# Autodesk Inventor assembly: Ensamble1
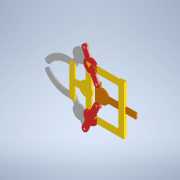
[picture p0: Inventor's stored thumbnail of the model, 180x180]
Saved by Autodesk Inventor 2021 (Build 250183000, 183)
## iProperties
Created: 2022-11-01
Part Number: Ensamble1
Document SubType Name: Assembly
Designer: USUARIO
Author: USUARIO
## Documents named in this file (6)
- C:\Users\USUARIO\Documents\Semestre8\Robótica\Proyecto-Rob\Piezas\Ensamble1.iam
- C:\Users\USUARIO\Documents\Semestre8\Robótica\Proyecto-Rob\Piezas\BaseGripper.ipt
- C:\Users\USUARIO\Documents\Semestre8\Robótica\Proyecto-Rob\Piezas\EslabonTransmisor.ipt
- C:\Users\USUARIO\Documents\Semestre8\Robótica\Proyecto-Rob\Piezas\Pinzas.ipt
- C:\Users\USUARIO\Documents\Semestre8\Robótica\Proyecto-Rob\Piezas\T.ipt
- C:\Users\USUARIO\Documents\Semestre8\Robótica\Proyecto-Rob\Piezas\Perno.ipt
## Components (12 placed, 5 different names)
1. BaseGripper:1 — Insert:1, Insert:2, Mate:1
2. EslabonTransmisor:1 — Insert:5, Insert:7
3. EslabonTransmisor:2 — Insert:6, Insert:8
4. Pinzas:1 — Insert:10, Insert:11
5. Pinzas:2 — Insert:12, Insert:13
6. T:1 — Insert:3, Insert:4, Mate:1
7. Perno:1 — Insert:3, Insert:5
8. Perno:2 — Insert:2, Insert:11
9. Perno:3 — Insert:1, Insert:13
10. Perno:4 — Insert:4, Insert:6
11. Perno:5 — Insert:7, Insert:12
12. Perno:6 — Insert:8, Insert:10
## Relationships (13: Insert 12, Mate 1)
- Insert:1: BaseGripper:1 ↔ Perno:3
- Insert:2: BaseGripper:1 ↔ Perno:2
- Insert:3: T:1 ↔ Perno:1
- Insert:4: T:1 ↔ Perno:4
- Insert:5: EslabonTransmisor:1 ↔ Perno:1
- Insert:6: EslabonTransmisor:2 ↔ Perno:4
- Insert:7: EslabonTransmisor:1 ↔ Perno:5
- Insert:8: EslabonTransmisor:2 ↔ Perno:6
- Insert:10: Pinzas:1 ↔ Perno:6
- Insert:11: Pinzas:1 ↔ Perno:2
- Insert:12: Pinzas:2 ↔ Perno:5
- Insert:13: Pinzas:2 ↔ Perno:3
- Mate:1: BaseGripper:1 ↔ T:1
